# Autodesk Inventor assembly: BackupNanoCase
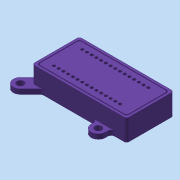
[picture p0: Inventor's stored thumbnail of the model, 180x180]
Saved by Autodesk Inventor 2017 (Build 210142000, 142)
## iProperties
Created: 2018-02-21
Part Number: BackupNanoCase
Document SubType Name: Assembly
Designer: Derek Wider
Author: Derek Wider
## Documents named in this file (4)
- D:\Projects\Submarine-project\CAD\midships\ElectronicsSection\BackupNanoCase.iam
- D:\Projects\Submarine-project\CAD\midships\ElectronicsSection\BackupNanoCasePart1.ipt
- D:\Projects\Submarine-project\CAD\midships\ElectronicsSection\BackupNanoCasePart2.ipt
- D:\Projects\Submarine-project\CAD\midships\ElectronicsSection\ArduinoNanoNoPins.iam
## Components (3 placed, 3 different names)
1. BackupNanoCasePart1:1 — Mate:2, Mate:3, Mate:4
2. BackupNanoCasePart2:1 — Flush:1, Mate:1, Angle:1, Mate:2, Mate:3, Mate:4
3. ArduinoNanoNoPins:1 [sub-assembly] — Flush:1, Mate:1, Angle:1
## Relationships (6: Mate 4, Flush 1, Angle 1)
- Flush:1 (-3.175 mm): BackupNanoCasePart2:1 ↔ ArduinoNanoNoPins:1
- Mate:1: BackupNanoCasePart2:1 ↔ ArduinoNanoNoPins:1
- Angle:1 (0 deg): BackupNanoCasePart2:1 ↔ ArduinoNanoNoPins:1
- Mate:2: BackupNanoCasePart1:1 ↔ BackupNanoCasePart2:1
- Mate:3 (0.3175 mm): BackupNanoCasePart1:1 ↔ BackupNanoCasePart2:1
- Mate:4 (0.3175 mm): BackupNanoCasePart1:1 ↔ BackupNanoCasePart2:1
